# Autodesk Inventor assembly: 360 Camera
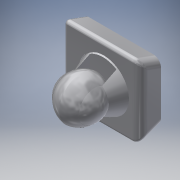
[picture p0: Inventor's stored thumbnail of the model, 180x180]
Saved by Autodesk Inventor 2017 (Build 210142000, 142)
## iProperties
Created: 2020-02-20
Part Number: 360 Camera
Document SubType Name: Assembly
Designer: S346852600
Author: S346852600
## Documents named in this file (5)
- \\ad.ocdsb.ca\studenthome\3\S338674153\FRC 2020\FullRobotRefactor\Parts\360 Camera.iam
- \\ad.ocdsb.ca\studenthome\3\S338674153\FRC 2020\FullRobotRefactor\Parts\2nd base.ipt
- \\ad.ocdsb.ca\studenthome\3\S338674153\FRC 2020\FullRobotRefactor\Parts\1st base.ipt
- \\ad.ocdsb.ca\studenthome\3\S338674153\FRC 2020\FullRobotRefactor\Parts\camera.ipt
- \\ad.ocdsb.ca\studenthome\3\S338674153\FRC 2020\FullRobotRefactor\Parts\camera side 2.ipt
## Components (5 placed, 4 different names)
1. 2nd base:1 — Mate:2, Mate:7, Mate:8
2. 1st base:1 — Mate:2, Flush:1, Mate:4, Mate:5, Flush:2, Mate:6, Mate:7, Mate:8, Mate:9
3. camera:1 — Mate:10, Mate:11
4. camera side 2:2 — Flush:1, Mate:4, Mate:9, Mate:10, Mate:11
5. camera side 2:3 — Mate:5, Flush:2, Mate:6
## Relationships (11: Mate 9, Flush 2)
- Mate:2: 2nd base:1 ↔ 1st base:1
- Flush:1: 1st base:1 ↔ camera side 2:2
- Mate:4: 1st base:1 ↔ camera side 2:2
- Mate:5: 1st base:1 ↔ camera side 2:3
- Flush:2: 1st base:1 ↔ camera side 2:3
- Mate:6: 1st base:1 ↔ camera side 2:3
- Mate:7: 2nd base:1 ↔ 1st base:1
- Mate:8: 2nd base:1 ↔ 1st base:1
- Mate:9: 1st base:1 ↔ camera side 2:2
- Mate:10: camera:1 ↔ camera side 2:2
- Mate:11: camera:1 ↔ camera side 2:2
